# Autodesk Inventor assembly: ASY Disk Micro filter old version
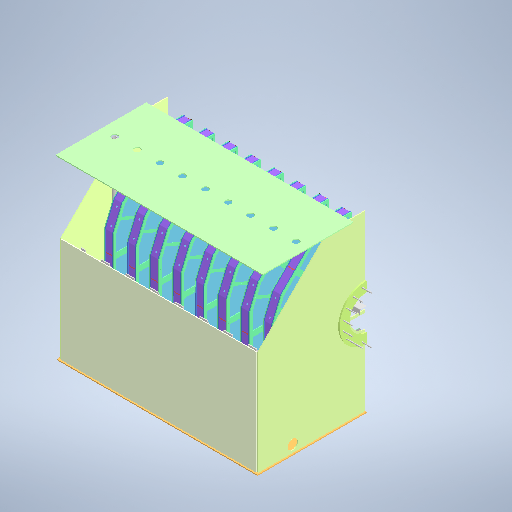
[picture p0: Inventor's stored thumbnail of the model, 512x512]
Saved by Autodesk Inventor 2025 (Build 290162010, 162A)
## iProperties
Created: 2023-08-31
Part Number: ASY Disk Micro filter old version
Document SubType Name: Assembly
Designer: admin
Stock Number: Дисковый_Фильтр
Author: admin
## Documents named in this file (29)
- C:\Users\pokla\Documents\Inventor\ДФО\ДМФ\DMF-Disk-Micro-Filter\DMF old version\ASY 000 ДМФ Disk Micro filter old version.iam
- C:\Users\pokla\Documents\Inventor\ДФО\ДМФ\DMF-Disk-Micro-Filter\DMF old version\Left wall.ipt
- C:\Users\pokla\Documents\Inventor\ДФО\ДМФ\DMF-Disk-Micro-Filter\DMF old version\Wall right.ipt
- C:\Users\pokla\Documents\Inventor\ДФО\ДМФ\DMF-Disk-Micro-Filter\DMF old version\DF1.03 Wall bottom.ipt
- C:\Users\pokla\Documents\Inventor\ДФО\ДМФ\DMF-Disk-Micro-Filter\DMF old version\DF1.04 Wall face.ipt
- C:\Users\pokla\Documents\Inventor\ДФО\ДМФ\DMF-Disk-Micro-Filter\DMF old version\ыASY xDF frame.iam
- C:\Users\pokla\Documents\Inventor\ДФО\ДМФ\DMF-Disk-Micro-Filter\DMF old version\ДМФ 021 кольцо прижимное нос.ipt
- C:\Users\pokla\Documents\Inventor\ДФО\ДМФ\DMF-Disk-Micro-Filter\DMF old version\ДМФ 000 размеры.ipt
- C:\Users\pokla\Documents\Inventor\ДФО\ДМФ\DMF-Disk-Micro-Filter\DMF old version\ASY ДМФ 030 кольцо со шпильками корма.iam
- C:\Users\pokla\Documents\Inventor\ДФО\ДМФ\DMF-Disk-Micro-Filter\DMF old version\ДМФ 032 крышка Нос.ipt
- C:\Users\pokla\Documents\Inventor\ДФО\ДМФ\DMF-Disk-Micro-Filter\DMF old version\ASY ДМФ 0100 Барабан.iam
- C:\Users\pokla\Documents\Inventor\ДФО\ДМФ\DMF-Disk-Micro-Filter\DMF old version\ДМФ 091 Постель НОС.ipt
- C:\Users\pokla\Documents\Inventor\ДФО\ДМФ\DMF-Disk-Micro-Filter\DMF old version\ASY ДМФ 040 кольцо под шпильки КОРМА.iam
- C:\Users\pokla\Documents\Inventor\ДФО\ДМФ\DMF-Disk-Micro-Filter\DMF old version\ДМФ 022 кольцо прижимное корма.ipt
- C:\Users\pokla\Documents\Inventor\ДФО\ДМФ\DMF-Disk-Micro-Filter\DMF old version\ДМФ 093 Постель КОРМА.ipt
- C:\Users\pokla\Documents\Inventor\ДФО\ДМФ\DMF-Disk-Micro-Filter\DMF old version\ДМФ 092 Коромысло КОРМА.ipt
- C:\Users\pokla\Documents\Inventor\ДФО\ДМФ\DMF-Disk-Micro-Filter\DMF old version\ДМФ 055 труба илоотвода.ipt
- C:\Users\pokla\Documents\Inventor\ДФО\ДМФ\DMF-Disk-Micro-Filter\DMF old version\ДМФ 033 держатель лотка.ipt
- C:\Users\pokla\Documents\Inventor\ДФО\ДМФ\DMF-Disk-Micro-Filter\DMF old version\ASY ДМФ лоток 050 илоотвод.iam
- C:\Users\pokla\Documents\Inventor\ДФО\ДМФ\DMF-Disk-Micro-Filter\DMF old version\ДМФ 092 Коромысло НОС.ipt
- C:\Users\pokla\Documents\Inventor\ДФО\ДМФ\DMF-Disk-Micro-Filter\DMF old version\ДМФ 011 Стенка Корма ЛЕВ.ipt
- C:\Users\pokla\Documents\Inventor\ДФО\ДМФ\DMF-Disk-Micro-Filter\DMF old version\ДМФ 012 Стенка Корма ПРАВ.ipt
- C:\Users\pokla\Documents\Inventor\ДФО\ДМФ\DMF-Disk-Micro-Filter\DMF old version\ДМФ 014 Стенка Нос ЛЕВ.ipt
- C:\Users\pokla\Documents\Inventor\ДФО\ДМФ\DMF-Disk-Micro-Filter\DMF old version\ДМФ 015 Стенка Нос ПРАВ.ipt
- C:\Users\pokla\Documents\Inventor\ДФО\ДМФ\DMF-Disk-Micro-Filter\DMF old version\ДМФ 066 Гребенка.ipt
- C:\Users\pokla\Documents\Inventor\ДФО\ДМФ\DMF-Disk-Micro-Filter\DMF old version\ДМФ 025 кольцо прижимное корма наружное.ipt
- C:\Users\pokla\Documents\Inventor\ДФО\ДМФ\DMF-Disk-Micro-Filter\DMF old version\ASY ДМФ 070 кольцо под шпильки КОРМА наружное.iam
- C:\Users\pokla\Documents\Inventor\ДФО\ДМФ\DMF-Disk-Micro-Filter\DMF old version\ДМФ 067 крышка.ipt
- C:\Users\pokla\Documents\Inventor\ДФО\ДМФ\DMF-Disk-Micro-Filter\DMF old version\ДМФ 081 труба форсунки.ipt
## Components (28 placed, 28 different names)
1. ДМФ 000 размеры.ipt:1
2. Left wall.ipt:1 — Flush:3, Flush:4, Mate:1, Flush:6, Flush:7, Flush:9, Mate:4, Flush:16, Rotational:12, Rigid:9, Rigid:12
3. Wall right.ipt:1 — Flush:3, Mate:2, Flush:8, Mate:22, Rigid:14, Flush:23, Flush:24
4. DF1.03 Wall bottom.ipt:1 — Mate:1, Mate:2, Flush:6, Flush:7, Flush:8, Mate:3, Flush:11, Mate:5, Mate:24
5. DF1.04 Wall face.ipt:1 — Flush:9, Mate:3, Mate:4, Flush:10, Angle:1
6. ыASY xDF frame.iam:1 [sub-assembly] — Flush:15, Flush:13, Flush:14, Mate:5
7. ДМФ 021 кольцо прижимное нос.ipt:1 — Rotational:12, Mate:13, Rotational:14
8. ASY ДМФ 030 кольцо со шпильками корма.iam:1 [sub-assembly] — Flush:16, Rigid:9
9. ДМФ 032 крышка Нос.ipt:1 — Mate:16, Rigid:8, Rigid:12
10. ASY ДМФ 0100 Барабан.iam:1 [sub-assembly] — Rotational:15
11. ДМФ 091 Постель НОС.ipt:1 — Flush:17, Rotational:14, Rigid:10, Rotational:15
12. ASY ДМФ 040 кольцо под шпильки КОРМА.iam:1 [sub-assembly] — Mate:14, Rigid:13
13. ДМФ 022 кольцо прижимное корма.ipt:1 — Flush:18, Rigid:11, Rigid:13
14. ДМФ 093 Постель КОРМА.ipt:1 — Mate:15, Rigid:3, Rigid:11
15. ДМФ 092 Коромысло КОРМА.ipt:1 — Rigid:3
16. ДМФ 055 труба илоотвода.ipt:1 — Rigid:8, Tangent:1
17. ДМФ 033 держатель лотка.ipt:1 — Mate:16, Mate:17, Tangent:1, Mate:23
18. ASY ДМФ лоток 050 илоотвод.iam:1 [sub-assembly] — Mate:22, Mate:23
19. ДМФ 092 Коромысло НОС.ipt:1 — Rigid:10
20. ДМФ 011 Стенка Корма ЛЕВ.ipt:1
21. ДМФ 012 Стенка Корма ПРАВ.ipt:1
22. ДМФ 014 Стенка Нос ЛЕВ.ipt:1
23. ДМФ 015 Стенка Нос ПРАВ.ipt:1
24. ДМФ 066 Гребенка.ipt:1 — Flush:22, Angle:1, Mate:24
25. ДМФ 025 кольцо прижимное корма наружное.ipt:1 — Rigid:14, Rigid:15
26. ASY ДМФ 070 кольцо под шпильки КОРМА наружное.iam:1 [sub-assembly] — Rigid:15
27. ДМФ 067 крышка.ipt:1 — Flush:23, Flush:24, Flush:25, Rotational:16
28. ДМФ 081 труба форсунки.ipt:1 — Flush:25, Rotational:16
## Relationships (48: Flush 19, Mate 14, WeldJoint 9, RevoluteJoint 4, Tangent 1, Angle 1)
- Flush:3: Left wall.ipt:1 ↔ Wall right.ipt:1
- Flush:4: Left wall.ipt:1
- Mate:1: Left wall.ipt:1 ↔ DF1.03 Wall bottom.ipt:1
- Mate:2: Wall right.ipt:1 ↔ DF1.03 Wall bottom.ipt:1
- Flush:6 (15 mm): Left wall.ipt:1 ↔ DF1.03 Wall bottom.ipt:1
- Flush:7 (25 mm): Left wall.ipt:1 ↔ DF1.03 Wall bottom.ipt:1
- Flush:8 (15 mm): Wall right.ipt:1 ↔ DF1.03 Wall bottom.ipt:1
- Flush:9: Left wall.ipt:1 ↔ DF1.04 Wall face.ipt:1
- Mate:3: DF1.03 Wall bottom.ipt:1 ↔ DF1.04 Wall face.ipt:1
- Mate:4: Left wall.ipt:1 ↔ DF1.04 Wall face.ipt:1
- Flush:10: DF1.04 Wall face.ipt:1
- Flush:11: DF1.03 Wall bottom.ipt:1
- [Flush]: ыASY xDF frame.iam:1
- Flush:15: ыASY xDF frame.iam:1
- Flush:13: ыASY xDF frame.iam:1
- Flush:14: ыASY xDF frame.iam:1
- Mate:5: DF1.03 Wall bottom.ipt:1 ↔ ыASY xDF frame.iam:1
- Flush:16: Left wall.ipt:1 ↔ ASY ДМФ 030 кольцо со шпильками корма.iam:1
- Rotational:12 [RevoluteJoint]: Left wall.ipt:1 ↔ ДМФ 021 кольцо прижимное нос.ipt:1
- Mate:13: ДМФ 021 кольцо прижимное нос.ipt:1
- Flush:17: ДМФ 091 Постель НОС.ipt:1
- Mate:14: ASY ДМФ 040 кольцо под шпильки КОРМА.iam:1
- Flush:18: ДМФ 022 кольцо прижимное корма.ipt:1
- Mate:15: ДМФ 093 Постель КОРМА.ipt:1
- Rigid:3 [WeldJoint]: ДМФ 093 Постель КОРМА.ipt:1 ↔ ДМФ 092 Коромысло КОРМА.ipt:1
- [Mate]: ASY ДМФ лоток 050 илоотвод.iam:1
- Mate:16: ДМФ 032 крышка Нос.ipt:1 ↔ ДМФ 033 держатель лотка.ipt:1
- Mate:17: ДМФ 033 держатель лотка.ipt:1
- Rigid:8 [WeldJoint]: ДМФ 032 крышка Нос.ipt:1 ↔ ДМФ 055 труба илоотвода.ipt:1
- Rigid:9 [WeldJoint]: Left wall.ipt:1 ↔ ASY ДМФ 030 кольцо со шпильками корма.iam:1
- Tangent:1: ДМФ 055 труба илоотвода.ipt:1 ↔ ДМФ 033 держатель лотка.ipt:1
- Mate:22: Wall right.ipt:1 ↔ ASY ДМФ лоток 050 илоотвод.iam:1
- Mate:23: ДМФ 033 держатель лотка.ipt:1 ↔ ASY ДМФ лоток 050 илоотвод.iam:1
- Rotational:14 [RevoluteJoint]: ДМФ 021 кольцо прижимное нос.ipt:1 ↔ ДМФ 091 Постель НОС.ipt:1
- Rigid:10 [WeldJoint]: ДМФ 091 Постель НОС.ipt:1 ↔ ДМФ 092 Коромысло НОС.ipt:1
- Rotational:15 [RevoluteJoint]: ASY ДМФ 0100 Барабан.iam:1 ↔ ДМФ 091 Постель НОС.ipt:1
- Rigid:11 [WeldJoint]: ДМФ 022 кольцо прижимное корма.ipt:1 ↔ ДМФ 093 Постель КОРМА.ipt:1
- Rigid:12 [WeldJoint]: Left wall.ipt:1 ↔ ДМФ 032 крышка Нос.ipt:1
- Flush:22: ДМФ 066 Гребенка.ipt:1
- Angle:1 (180 deg): DF1.04 Wall face.ipt:1 ↔ ДМФ 066 Гребенка.ipt:1
- Mate:24: DF1.03 Wall bottom.ipt:1 ↔ ДМФ 066 Гребенка.ipt:1
- Rigid:13 [WeldJoint]: ASY ДМФ 040 кольцо под шпильки КОРМА.iam:1 ↔ ДМФ 022 кольцо прижимное корма.ipt:1
- Rigid:14 [WeldJoint]: Wall right.ipt:1 ↔ ДМФ 025 кольцо прижимное корма наружное.ipt:1
- Rigid:15 [WeldJoint]: ДМФ 025 кольцо прижимное корма наружное.ipt:1 ↔ ASY ДМФ 070 кольцо под шпильки КОРМА наружное.iam:1
- Flush:23: Wall right.ipt:1 ↔ ДМФ 067 крышка.ipt:1
- Flush:24 (-50 mm): Wall right.ipt:1 ↔ ДМФ 067 крышка.ipt:1
- Flush:25: ДМФ 067 крышка.ipt:1 ↔ ДМФ 081 труба форсунки.ipt:1
- Rotational:16 [RevoluteJoint]: ДМФ 067 крышка.ipt:1 ↔ ДМФ 081 труба форсунки.ipt:1
